# Autodesk Inventor assembly: робот - сборка фулл
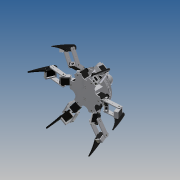
[picture p0: Inventor's stored thumbnail of the model, 180x180]
Saved by Autodesk Inventor 2020 (Build 240168000, 168)
## iProperties
Created: 2019-09-07
Part Number: робот - сборка фулл
Material: Типовые
Document SubType Name: Assembly
Designer: Iliga
Author: Iliga
## Documents named in this file (28)
- F:\GrabCAD\Robot\робот - сборка фулл.iam
- F:\GrabCAD\Robot\тело.ipt
- F:\GrabCAD\Robot\левая лапа - сборка.iam
- F:\GrabCAD\Robot\крепление2.ipt
- F:\GrabCAD\Robot\крепление-стенки.ipt
- F:\GrabCAD\Robot\полочка.ipt
- F:\GrabCAD\Robot\1.ipt
- F:\GrabCAD\Robot\Camera OV7670.iam
- F:\GrabCAD\Robot\28BYJ-48 – 5V Stepper Motor.ipt
- F:\GrabCAD\Robot\Крепление_двигатель малый.ipt
- F:\GrabCAD\Robot\Крепление_база.ipt
- F:\GrabCAD\Robot\Деталь1.ipt
- F:\GrabCAD\Robot\EN ISO 7045 - M4 x 8 - 4.8 - H(1).ipt
- F:\GrabCAD\Robot\EN ISO 7045 - M2 x 6 - 4.8 - H(1).ipt
- F:\GrabCAD\Robot\EN ISO 7045 - M1,6 x 4 - 4.8 - H(1).ipt
- F:\GrabCAD\Robot\EN ISO 7045 - M6 x 8 - 4.8 - H(1).ipt
- F:\GrabCAD\Robot\MP1584 Regulador.ipt
- F:\GrabCAD\Robot\Крепление Меги.ipt
- F:\GrabCAD\Robot\arduinoMegaDetailed.ipt
- F:\GrabCAD\Robot\Крепление батареек.ipt
- F:\GrabCAD\Robot\AAA_SIZE_BATTERY_CELL.ipt
- F:\GrabCAD\Robot\Bluetooth adapter крышка.ipt
- F:\GrabCAD\Robot\DC-DC корпус.ipt
- F:\GrabCAD\Robot\Bluetooth adapter корпус.ipt
- F:\GrabCAD\Robot\HM10.iam
- F:\GrabCAD\Robot\EN ISO 7045 - M3 x 6 - 4.8 - H(1).ipt
- F:\GrabCAD\Robot\ULN2003.ipt
- F:\GrabCAD\Robot\крепление_драйвера.ipt
## Components (135 placed, 25 different names)
1. лапа:1 [sub-assembly] — Совмещение:92, Совмещение:97, Совмещение:173, Совмещение:179
2. лапа:2 [sub-assembly] — Совмещение:89, Совмещение:91, Совмещение:175
3. лапа:3 [sub-assembly] — Совмещение:90, Совмещение:96
4. лапа:4 [sub-assembly] — Совмещение:159, Совмещение:160, Совмещение:178
5. лапа:5 [sub-assembly] — Совмещение:161, Совмещение:163
6. лапа:6 [sub-assembly] — Совмещение:162, Совмещение:164, Совмещение:176
7. крепление-стенки:1 — Совмещение:86, Совмещение:87, Совмещение:88, Совмещение:126, Совмещение:127, Совмещение:128
8. крепление2:1 — Совмещение:86, Совмещение:87, Совмещение:88, Совмещение:89, Совмещение:90, Совмещение:91, Совмещение:92, Совмещение:96, Совмещение:97, Совмещение:166, Совмещение:167, Совмещение:168, Совмещение:169, Совмещение:170, Совмещение:171, Совмещение:172, Допуск симметричности:1
9. тело основа:1 — Совмещение:49, Заподлицо:1, Касательность:1, Совмещение:118, Совмещение:132, Совмещение:184, Совмещение:185, Совмещение:186, Совмещение:187
10. тело основа:2 — Совмещение:49, Заподлицо:1, Касательность:1, Совмещение:120, Совмещение:121, Совмещение:122, Совмещение:123
11. тело основа:3 — Совмещение:120, Совмещение:121, Совмещение:122, Заподлицо:2, Совмещение:126, Совмещение:127, Совмещение:128, Совмещение:159, Совмещение:160, Совмещение:161, Совмещение:162, Совмещение:163, Совмещение:164, Допуск симметричности:1, Совмещение:173, Совмещение:175, Совмещение:176, Совмещение:178, Совмещение:179, Совмещение:180, Совмещение:181, Совмещение:182, Совмещение:183
12. полочка:1 — Совмещение:118, Совмещение:123, Заподлицо:2, Заподлицо:4, Совмещение:136, Совмещение:137, Совмещение:138, Совмещение:140, Совмещение:141, Совмещение:142, Совмещение:143, Совмещение:144, Совмещение:149, Совмещение:150, Совмещение:151, Совмещение:152, Совмещение:225, Совмещение:238, Совмещение:309, Совмещение:373, Совмещение:378, Совмещение:379, Совмещение:392, Совмещение:397, Совмещение:398, Совмещение:399, Совмещение:400, Совмещение:401, Совмещение:402, Совмещение:403, Совмещение:404, Совмещение:405, Совмещение:406, Совмещение:407, Совмещение:408, Совмещение:409, Совмещение:410, Совмещение:411, Совмещение:412, Совмещение:413, Совмещение:429, Совмещение:430, Совмещение:431, Совмещение:447, Совмещение:448, Совмещение:449, Совмещение:465, Совмещение:466, Совмещение:467
13. Camera OV7670:1 [sub-assembly] — Совмещение:156, Совмещение:165
14. 28BYJ-48 – 5V Stepper Motor:1 — Совмещение:131, Совмещение:132, Заподлицо:4, Совмещение:133, Совмещение:134, Совмещение:135, Совмещение:153, Совмещение:154, Совмещение:155
15. Крепление_двигатель малый:1 — Совмещение:133, Совмещение:134, Совмещение:135
16. Крепление:1 — Совмещение:137, Совмещение:141, Совмещение:142
17. Крепление:2 — Совмещение:136, Совмещение:138, Совмещение:140
18. Крепление:3 — Совмещение:144, Совмещение:151, Совмещение:152
19. Крепление:4 — Совмещение:143, Совмещение:149, Совмещение:150
20. Деталь1:1 — Совмещение:153, Совмещение:154, Совмещение:155, Совмещение:156, Совмещение:165
21. BS EN ISO 7045 H - метрическая M2 x 6 - 4.8 - H:9 — Заподлицо:8, Заподлицо:10
22. BS EN ISO 7045 H - метрическая M2 x 6 - 4.8 - H:10 — Заподлицо:8
23. BS EN ISO 7045 H - метрическая M2 x 6 - 4.8 - H:11 — Заподлицо:9, Заподлицо:10
24. BS EN ISO 7045 H - метрическая M2 x 6 - 4.8 - H:12 — Заподлицо:9
25. BS EN ISO 7045 H - метрическая M2 x 6 - 4.8 - H:13
26. BS EN ISO 7045 H - метрическая M2 x 6 - 4.8 - H:14
27. BS EN ISO 7045 H - метрическая M2 x 6 - 4.8 - H:15
28. BS EN ISO 7045 H - метрическая M2 x 6 - 4.8 - H:16
29. BS EN ISO 7045 H - метрическая M6 x 8 - 4.8 - H:1 — Совмещение:184, Совмещение:185
30. BS EN ISO 7045 H - метрическая M6 x 8 - 4.8 - H:2 — Совмещение:186, Совмещение:187
31. MP1584 Regulador:1 — Совмещение:208, Совмещение:209, Совмещение:210
32. Крепление Меги:1 — Совмещение:188, Совмещение:189, Совмещение:190, Совмещение:191, Совмещение:192, Совмещение:193
33. arduinoMegaDetailed:1 — Совмещение:188, Совмещение:189, Совмещение:190, Совмещение:239, Совмещение:240, Совмещение:241, Совмещение:242
34. Крепление батареек:1 — Совмещение:194, Совмещение:195, Совмещение:196, Совмещение:197, Совмещение:198, Совмещение:199, Совмещение:200, Совмещение:201
35. AAA_SIZE_BATTERY_CELL:1 — Совмещение:194, Заподлицо:15, Совмещение:198
36. AAA_SIZE_BATTERY_CELL:2 — Совмещение:195, Заподлицо:14, Заподлицо:15
37. AAA_SIZE_BATTERY_CELL:3 — Совмещение:196, Заподлицо:13, Заподлицо:14
38. AAA_SIZE_BATTERY_CELL:4 — Совмещение:197, Заподлицо:13
39. DC-DC крышка:1 — Совмещение:211, Совмещение:212, Заподлицо:16
40. DC-DC корпус:1 — Совмещение:208, Совмещение:209, Совмещение:210, Совмещение:211, Совмещение:212, Заподлицо:16, Совмещение:213, Совмещение:214, Совмещение:215, Совмещение:216, Совмещение:217, Совмещение:218, Совмещение:219, Совмещение:220, Совмещение:221, Совмещение:222, Совмещение:223, Совмещение:224
41. Крепление:13 — Совмещение:213, Совмещение:214, Совмещение:215, Совмещение:225
42. Крепление:14 — Совмещение:216, Совмещение:217, Совмещение:218
43. Крепление:15 — Совмещение:219, Совмещение:220, Совмещение:221, Совмещение:407, Совмещение:408
44. Крепление:16 — Совмещение:222, Совмещение:223, Совмещение:224
45. DC-DC корпус:2 — Совмещение:228, Совмещение:229, Совмещение:230, Заподлицо:17, Совмещение:231, Совмещение:232, Совмещение:233, Совмещение:234, Совмещение:235
46. DC-DC крышка:2 — Заподлицо:17, Совмещение:231, Совмещение:232
47. HM10:1 [sub-assembly] — Совмещение:228, Совмещение:229, Совмещение:230
48. BS EN ISO 7045 H - метрическая M3 x 6 - 4.8 - H:1 — Совмещение:241, Совмещение:242
49. BS EN ISO 7045 H - метрическая M3 x 6 - 4.8 - H:2 — Совмещение:239, Совмещение:240
50. ULN2003:1 — Совмещение:244, Совмещение:245, Совмещение:246
51. крепление_драйвера:1 — Совмещение:244, Совмещение:245, Совмещение:246, Совмещение:380, Совмещение:381, Совмещение:382, Совмещение:383, Совмещение:384, Совмещение:385, Совмещение:386, Совмещение:387, Совмещение:388, Совмещение:389, Совмещение:390, Совмещение:391
52. Крепление:21 — Совмещение:380, Совмещение:381, Совмещение:382
53. MP1584 Regulador:2
54. DC-DC корпус:3
55. Крепление:25
56. Крепление:26
57. Крепление:27 — Совмещение:309, Совмещение:409, Совмещение:410
58. Крепление:28
59. MP1584 Regulador:4
60. DC-DC корпус:5
61. Крепление:33
62. Крепление:34
63. Крепление:35 — Совмещение:411, Совмещение:412, Совмещение:413
64. Крепление:36
65. MP1584 Regulador:7
66. DC-DC корпус:8
67. Крепление:45
68. Крепление:46
69. Крепление:47 — Совмещение:405, Совмещение:406
70. Крепление:48 — Совмещение:373
71. Крепление:49 — Совмещение:383, Совмещение:384, Совмещение:385, Совмещение:392, Совмещение:400, Совмещение:401
72. Крепление:50 — Совмещение:386, Совмещение:387, Совмещение:388
73. Крепление:51 — Совмещение:389, Совмещение:390, Совмещение:391
74. MP1584 Regulador:8
75. DC-DC корпус:9
76. Крепление:52
77. Крепление:53
78. Крепление:54 — Совмещение:429, Совмещение:430, Совмещение:431
79. Крепление:55
80. MP1584 Regulador:9
81. DC-DC корпус:10
82. Крепление:56 — Совмещение:447
83. Крепление:57 — Совмещение:448, Совмещение:449
84. Крепление:58
85. Крепление:59
86. MP1584 Regulador:10
87. DC-DC корпус:11
88. Крепление:60
89. Крепление:61
90. Крепление:62 — Совмещение:465, Совмещение:466, Совмещение:467
91. Крепление:63
92. BS EN ISO 7045 H - метрическая M4 x 8 - 4.8 - H:1 — Совмещение:166, Совмещение:167
93. BS EN ISO 7045 H - метрическая M4 x 8 - 4.8 - H:2
94. BS EN ISO 7045 H - метрическая M4 x 8 - 4.8 - H:3
95. BS EN ISO 7045 H - метрическая M4 x 8 - 4.8 - H:4
96. BS EN ISO 7045 H - метрическая M4 x 8 - 4.8 - H:5
97. BS EN ISO 7045 H - метрическая M4 x 8 - 4.8 - H:6
98. BS EN ISO 7045 H - метрическая M2 x 6 - 4.8 - H:1 — Заподлицо:5, Заподлицо:6, Совмещение:171
99. BS EN ISO 7045 H - метрическая M2 x 6 - 4.8 - H:2 — Заподлицо:5, Совмещение:169, Совмещение:172
100. BS EN ISO 7045 H - метрическая M2 x 6 - 4.8 - H:4 — Заподлицо:6, Заподлицо:7, Совмещение:168
101. BS EN ISO 7045 H - метрическая M2 x 6 - 4.8 - H:3 — Заподлицо:7, Совмещение:170
102. BS EN ISO 7045 H - метрическая M2 x 6 - 4.8 - H:5
103. BS EN ISO 7045 H - метрическая M2 x 6 - 4.8 - H:6
104. BS EN ISO 7045 H - метрическая M2 x 6 - 4.8 - H:7
105. BS EN ISO 7045 H - метрическая M2 x 6 - 4.8 - H:8
106. BS EN ISO 7045 H - метрическая M1,6 x 4 - 4.8 - H:1 — Заподлицо:11, Совмещение:181
107. BS EN ISO 7045 H - метрическая M1,6 x 4 - 4.8 - H:3 — Заподлицо:11, Заподлицо:12, Совмещение:180
108. BS EN ISO 7045 H - метрическая M1,6 x 4 - 4.8 - H:2 — Заподлицо:12, Совмещение:182, Совмещение:183
109. BS EN ISO 7045 H - метрическая M1,6 x 4 - 4.8 - H:4
110. BS EN ISO 7045 H - метрическая M1,6 x 4 - 4.8 - H:5
111. BS EN ISO 7045 H - метрическая M1,6 x 4 - 4.8 - H:6
112. BS EN ISO 7045 H - метрическая M1,6 x 4 - 4.8 - H:7
113. BS EN ISO 7045 H - метрическая M1,6 x 4 - 4.8 - H:8
114. BS EN ISO 7045 H - метрическая M1,6 x 4 - 4.8 - H:9
115. BS EN ISO 7045 H - метрическая M1,6 x 4 - 4.8 - H:10
116. BS EN ISO 7045 H - метрическая M1,6 x 4 - 4.8 - H:11
117. BS EN ISO 7045 H - метрическая M1,6 x 4 - 4.8 - H:12
118. BS EN ISO 7045 H - метрическая M1,6 x 4 - 4.8 - H:13
119. BS EN ISO 7045 H - метрическая M1,6 x 4 - 4.8 - H:14
120. BS EN ISO 7045 H - метрическая M1,6 x 4 - 4.8 - H:15
121. BS EN ISO 7045 H - метрическая M1,6 x 4 - 4.8 - H:16
122. BS EN ISO 7045 H - метрическая M1,6 x 4 - 4.8 - H:17
123. BS EN ISO 7045 H - метрическая M1,6 x 4 - 4.8 - H:18
124. Крепление:5 — Совмещение:191, Совмещение:192, Совмещение:193, Совмещение:397, Совмещение:398, Совмещение:399
125. Крепление:6
126. Крепление:7
127. Крепление:8
128. Крепление:9 — Совмещение:199, Совмещение:200, Совмещение:201, Совмещение:402, Совмещение:403, Совмещение:404
129. Крепление:10
130. Крепление:11
131. Крепление:12
132. Крепление:17 — Совмещение:233, Совмещение:234, Совмещение:235, Совмещение:238, Совмещение:378, Совмещение:379
133. Крепление:18
134. Крепление:19
135. Крепление:20
## Component patterns: (6 elements, first: BS EN ISO 7045 H - метрическая M4 x 8 - 4.8 - H:1), (2 elements, first: BS EN ISO 7045 H - метрическая M2 x 6 - 4.8 - H:1 + BS EN ISO 7045 H - метрическая M2 x 6 - 4.8 - H:2 + BS EN ISO 7045 H - метрическая M2 x 6 - 4.8 - H:4 + BS EN ISO 7045 H - метрическая M2 x 6 - 4.8 - H:3), (6 elements, first: BS EN ISO 7045 H - метрическая M1,6 x 4 - 4.8 - H:1 + BS EN ISO 7045 H - метрическая M1,6 x 4 - 4.8 - H:3 + BS EN ISO 7045 H - метрическая M1,6 x 4 - 4.8 - H:2), (4 elements, first: Крепление:5), (4 elements, first: Крепление:9), (4 elements, first: Крепление:17)
## Relationships (265: Mate 247, Flush 16, Tangent 1, Symmetry 1)
- Совмещение:49 [Mate]: тело основа:1 ↔ тело основа:2
- Заподлицо:1 [Flush]: тело основа:1 ↔ тело основа:2
- Совмещение:86 [Mate]: крепление-стенки:1 ↔ крепление2:1
- Совмещение:87 [Mate]: крепление-стенки:1 ↔ крепление2:1
- Совмещение:88 [Mate]: крепление-стенки:1 ↔ крепление2:1
- Совмещение:89 [Mate]: лапа:2 ↔ крепление2:1
- Совмещение:90 [Mate]: лапа:3 ↔ крепление2:1
- Совмещение:91 [Mate]: лапа:2 ↔ крепление2:1
- Совмещение:92 [Mate]: лапа:1 ↔ крепление2:1
- Совмещение:96 [Mate]: лапа:3 ↔ крепление2:1
- Совмещение:97 [Mate]: лапа:1 ↔ крепление2:1
- Касательность:1 [Tangent]: тело основа:1 ↔ тело основа:2
- Совмещение:118 [Mate]: тело основа:1 ↔ полочка:1
- Совмещение:120 [Mate]: тело основа:2 ↔ тело основа:3
- Совмещение:121 [Mate]: тело основа:2 ↔ тело основа:3
- Совмещение:122 [Mate]: тело основа:2 ↔ тело основа:3
- Совмещение:123 [Mate]: тело основа:2 ↔ полочка:1
- Заподлицо:2 [Flush]: тело основа:3 ↔ полочка:1
- Совмещение:126 [Mate]: крепление-стенки:1 ↔ тело основа:3
- Совмещение:127 [Mate]: крепление-стенки:1 ↔ тело основа:3
- Совмещение:128 [Mate]: крепление-стенки:1 ↔ тело основа:3
- Совмещение:131 [Mate]: 28BYJ-48 – 5V Stepper Motor:1
- Совмещение:132 [Mate]: тело основа:1 ↔ 28BYJ-48 – 5V Stepper Motor:1
- Заподлицо:4 [Flush]: полочка:1 ↔ 28BYJ-48 – 5V Stepper Motor:1
- Совмещение:133 [Mate]: 28BYJ-48 – 5V Stepper Motor:1 ↔ Крепление_двигатель малый:1
- Совмещение:134 [Mate]: 28BYJ-48 – 5V Stepper Motor:1 ↔ Крепление_двигатель малый:1
- Совмещение:135 [Mate]: 28BYJ-48 – 5V Stepper Motor:1 ↔ Крепление_двигатель малый:1
- Совмещение:136 [Mate]: полочка:1 ↔ Крепление:2
- Совмещение:137 [Mate]: полочка:1 ↔ Крепление:1
- Совмещение:138 [Mate]: полочка:1 ↔ Крепление:2
- Совмещение:140 [Mate]: полочка:1 ↔ Крепление:2
- Совмещение:141 [Mate]: полочка:1 ↔ Крепление:1
- Совмещение:142 [Mate]: полочка:1 ↔ Крепление:1
- Совмещение:143 [Mate]: полочка:1 ↔ Крепление:4
- Совмещение:144 [Mate]: полочка:1 ↔ Крепление:3
- Совмещение:149 [Mate]: полочка:1 ↔ Крепление:4
- Совмещение:150 [Mate]: полочка:1 ↔ Крепление:4
- Совмещение:151 [Mate]: полочка:1 ↔ Крепление:3
- Совмещение:152 [Mate]: полочка:1 ↔ Крепление:3
- Совмещение:153 [Mate]: 28BYJ-48 – 5V Stepper Motor:1 ↔ Деталь1:1
- Совмещение:154 [Mate] (0.1 mm): 28BYJ-48 – 5V Stepper Motor:1 ↔ Деталь1:1
- Совмещение:155 [Mate]: 28BYJ-48 – 5V Stepper Motor:1 ↔ Деталь1:1
- Совмещение:156 [Mate]: Camera OV7670:1 ↔ Деталь1:1
- Совмещение:159 [Mate]: лапа:4 ↔ тело основа:3
- Совмещение:160 [Mate]: лапа:4 ↔ тело основа:3
- Совмещение:161 [Mate]: лапа:5 ↔ тело основа:3
- Совмещение:162 [Mate]: лапа:6 ↔ тело основа:3
- Совмещение:163 [Mate]: лапа:5 ↔ тело основа:3
- Совмещение:164 [Mate]: лапа:6 ↔ тело основа:3
- Совмещение:165 [Mate]: Camera OV7670:1 ↔ Деталь1:1
- Совмещение:166 [Mate]: крепление2:1 ↔ BS EN ISO 7045 H - метрическая M4 x 8 - 4.8 - H:1
- Совмещение:167 [Mate]: крепление2:1 ↔ BS EN ISO 7045 H - метрическая M4 x 8 - 4.8 - H:1
- Заподлицо:5 [Flush]: BS EN ISO 7045 H - метрическая M2 x 6 - 4.8 - H:1 ↔ BS EN ISO 7045 H - метрическая M2 x 6 - 4.8 - H:2
- Заподлицо:6 [Flush]: BS EN ISO 7045 H - метрическая M2 x 6 - 4.8 - H:1 ↔ BS EN ISO 7045 H - метрическая M2 x 6 - 4.8 - H:4
- Заподлицо:7 [Flush]: BS EN ISO 7045 H - метрическая M2 x 6 - 4.8 - H:4 ↔ BS EN ISO 7045 H - метрическая M2 x 6 - 4.8 - H:3
- Совмещение:168 [Mate]: крепление2:1 ↔ BS EN ISO 7045 H - метрическая M2 x 6 - 4.8 - H:4
- Совмещение:169 [Mate]: крепление2:1 ↔ BS EN ISO 7045 H - метрическая M2 x 6 - 4.8 - H:2
- Совмещение:170 [Mate]: крепление2:1 ↔ BS EN ISO 7045 H - метрическая M2 x 6 - 4.8 - H:3
- Совмещение:171 [Mate]: крепление2:1 ↔ BS EN ISO 7045 H - метрическая M2 x 6 - 4.8 - H:1
- Совмещение:172 [Mate]: крепление2:1 ↔ BS EN ISO 7045 H - метрическая M2 x 6 - 4.8 - H:2
- Допуск симметричности:1 [Symmetry]: крепление2:1 ↔ тело основа:3
- Заподлицо:8 [Flush]: BS EN ISO 7045 H - метрическая M2 x 6 - 4.8 - H:9 ↔ BS EN ISO 7045 H - метрическая M2 x 6 - 4.8 - H:10
- Заподлицо:9 [Flush]: BS EN ISO 7045 H - метрическая M2 x 6 - 4.8 - H:11 ↔ BS EN ISO 7045 H - метрическая M2 x 6 - 4.8 - H:12
- Заподлицо:10 [Flush]: BS EN ISO 7045 H - метрическая M2 x 6 - 4.8 - H:9 ↔ BS EN ISO 7045 H - метрическая M2 x 6 - 4.8 - H:11
- Совмещение:173 [Mate]: лапа:1 ↔ тело основа:3
- Совмещение:175 [Mate]: лапа:2 ↔ тело основа:3
- Совмещение:176 [Mate]: лапа:6 ↔ тело основа:3
- Совмещение:178 [Mate]: лапа:4 ↔ тело основа:3
- Совмещение:179 [Mate]: лапа:1 ↔ тело основа:3
- Заподлицо:11 [Flush]: BS EN ISO 7045 H - метрическая M1,6 x 4 - 4.8 - H:1 ↔ BS EN ISO 7045 H - метрическая M1,6 x 4 - 4.8 - H:3
- Заподлицо:12 [Flush]: BS EN ISO 7045 H - метрическая M1,6 x 4 - 4.8 - H:3 ↔ BS EN ISO 7045 H - метрическая M1,6 x 4 - 4.8 - H:2
- Совмещение:180 [Mate]: тело основа:3 ↔ BS EN ISO 7045 H - метрическая M1,6 x 4 - 4.8 - H:3
- Совмещение:181 [Mate]: тело основа:3 ↔ BS EN ISO 7045 H - метрическая M1,6 x 4 - 4.8 - H:1
- Совмещение:182 [Mate]: тело основа:3 ↔ BS EN ISO 7045 H - метрическая M1,6 x 4 - 4.8 - H:2
- Совмещение:183 [Mate]: тело основа:3 ↔ BS EN ISO 7045 H - метрическая M1,6 x 4 - 4.8 - H:2
- Совмещение:184 [Mate]: тело основа:1 ↔ BS EN ISO 7045 H - метрическая M6 x 8 - 4.8 - H:1
- Совмещение:185 [Mate]: тело основа:1 ↔ BS EN ISO 7045 H - метрическая M6 x 8 - 4.8 - H:1
- Совмещение:186 [Mate]: тело основа:1 ↔ BS EN ISO 7045 H - метрическая M6 x 8 - 4.8 - H:2
- Совмещение:187 [Mate]: тело основа:1 ↔ BS EN ISO 7045 H - метрическая M6 x 8 - 4.8 - H:2
- Совмещение:188 [Mate]: Крепление Меги:1 ↔ arduinoMegaDetailed:1
- Совмещение:189 [Mate]: Крепление Меги:1 ↔ arduinoMegaDetailed:1
- Совмещение:190 [Mate]: Крепление Меги:1 ↔ arduinoMegaDetailed:1
- Совмещение:191 [Mate]: Крепление Меги:1 ↔ Крепление:5
- Совмещение:192 [Mate]: Крепление Меги:1 ↔ Крепление:5
- Совмещение:193 [Mate]: Крепление Меги:1 ↔ Крепление:5
- Совмещение:194 [Mate]: Крепление батареек:1 ↔ AAA_SIZE_BATTERY_CELL:1
- Совмещение:195 [Mate]: Крепление батареек:1 ↔ AAA_SIZE_BATTERY_CELL:2
- Совмещение:196 [Mate]: Крепление батареек:1 ↔ AAA_SIZE_BATTERY_CELL:3
- Совмещение:197 [Mate]: Крепление батареек:1 ↔ AAA_SIZE_BATTERY_CELL:4
- Заподлицо:13 [Flush]: AAA_SIZE_BATTERY_CELL:3 ↔ AAA_SIZE_BATTERY_CELL:4
- Заподлицо:14 [Flush]: AAA_SIZE_BATTERY_CELL:2 ↔ AAA_SIZE_BATTERY_CELL:3
- Заподлицо:15 [Flush]: AAA_SIZE_BATTERY_CELL:1 ↔ AAA_SIZE_BATTERY_CELL:2
- Совмещение:198 [Mate]: Крепление батареек:1 ↔ AAA_SIZE_BATTERY_CELL:1
- Совмещение:199 [Mate]: Крепление батареек:1 ↔ Крепление:9
- Совмещение:200 [Mate]: Крепление батареек:1 ↔ Крепление:9
- Совмещение:201 [Mate]: Крепление батареек:1 ↔ Крепление:9
- Совмещение:208 [Mate]: MP1584 Regulador:1 ↔ DC-DC корпус:1
- Совмещение:209 [Mate]: MP1584 Regulador:1 ↔ DC-DC корпус:1
- Совмещение:210 [Mate]: MP1584 Regulador:1 ↔ DC-DC корпус:1
- Совмещение:211 [Mate]: DC-DC крышка:1 ↔ DC-DC корпус:1
- Совмещение:212 [Mate]: DC-DC крышка:1 ↔ DC-DC корпус:1
- Заподлицо:16 [Flush]: DC-DC крышка:1 ↔ DC-DC корпус:1
- Совмещение:213 [Mate]: DC-DC корпус:1 ↔ Крепление:13
- Совмещение:214 [Mate]: DC-DC корпус:1 ↔ Крепление:13
- Совмещение:215 [Mate]: DC-DC корпус:1 ↔ Крепление:13
- Совмещение:216 [Mate]: DC-DC корпус:1 ↔ Крепление:14
- Совмещение:217 [Mate]: DC-DC корпус:1 ↔ Крепление:14
- Совмещение:218 [Mate]: DC-DC корпус:1 ↔ Крепление:14
- Совмещение:219 [Mate]: DC-DC корпус:1 ↔ Крепление:15
- Совмещение:220 [Mate]: DC-DC корпус:1 ↔ Крепление:15
- Совмещение:221 [Mate]: DC-DC корпус:1 ↔ Крепление:15
- Совмещение:222 [Mate]: DC-DC корпус:1 ↔ Крепление:16
- Совмещение:223 [Mate]: DC-DC корпус:1 ↔ Крепление:16
- Совмещение:224 [Mate]: DC-DC корпус:1 ↔ Крепление:16
- Совмещение:225 [Mate]: полочка:1 ↔ Крепление:13
- Совмещение:228 [Mate]: DC-DC корпус:2 ↔ HM10:1
- Совмещение:229 [Mate]: DC-DC корпус:2 ↔ HM10:1
- Совмещение:230 [Mate]: DC-DC корпус:2 ↔ HM10:1
- Заподлицо:17 [Flush]: DC-DC корпус:2 ↔ DC-DC крышка:2
- Совмещение:231 [Mate]: DC-DC корпус:2 ↔ DC-DC крышка:2
- Совмещение:232 [Mate]: DC-DC корпус:2 ↔ DC-DC крышка:2
- Совмещение:233 [Mate]: DC-DC корпус:2 ↔ Крепление:17
- Совмещение:234 [Mate]: DC-DC корпус:2 ↔ Крепление:17
- Совмещение:235 [Mate]: DC-DC корпус:2 ↔ Крепление:17
- Совмещение:238 [Mate]: полочка:1 ↔ Крепление:17
- Совмещение:239 [Mate]: arduinoMegaDetailed:1 ↔ BS EN ISO 7045 H - метрическая M3 x 6 - 4.8 - H:2
- Совмещение:240 [Mate]: arduinoMegaDetailed:1 ↔ BS EN ISO 7045 H - метрическая M3 x 6 - 4.8 - H:2
- Совмещение:241 [Mate]: arduinoMegaDetailed:1 ↔ BS EN ISO 7045 H - метрическая M3 x 6 - 4.8 - H:1
- Совмещение:242 [Mate]: arduinoMegaDetailed:1 ↔ BS EN ISO 7045 H - метрическая M3 x 6 - 4.8 - H:1
- Совмещение:244 [Mate]: ULN2003:1 ↔ крепление_драйвера:1
- Совмещение:245 [Mate]: ULN2003:1 ↔ крепление_драйвера:1
- Совмещение:246 [Mate]: ULN2003:1 ↔ крепление_драйвера:1
- [Mate]: MP1584 Regulador:2 ↔ DC-DC корпус:3
- [Mate]: MP1584 Regulador:2 ↔ DC-DC корпус:3
- [Mate]: MP1584 Regulador:2 ↔ DC-DC корпус:3
- [Mate]: DC-DC корпус:3 ↔ Крепление:25
- [Mate]: DC-DC корпус:3 ↔ Крепление:25
- [Mate]: DC-DC корпус:3 ↔ Крепление:25
- [Mate]: DC-DC корпус:3 ↔ Крепление:26
- [Mate]: DC-DC корпус:3 ↔ Крепление:26
- [Mate]: DC-DC корпус:3 ↔ Крепление:26
- [Mate]: DC-DC корпус:3 ↔ Крепление:27
- [Mate]: DC-DC корпус:3 ↔ Крепление:27
- [Mate]: DC-DC корпус:3 ↔ Крепление:27
- [Mate]: DC-DC корпус:3 ↔ Крепление:28
- [Mate]: DC-DC корпус:3 ↔ Крепление:28
- [Mate]: DC-DC корпус:3 ↔ Крепление:28
- [Mate]: MP1584 Regulador:4 ↔ DC-DC корпус:5
- [Mate]: MP1584 Regulador:4 ↔ DC-DC корпус:5
- [Mate]: MP1584 Regulador:4 ↔ DC-DC корпус:5
- [Mate]: DC-DC корпус:5 ↔ Крепление:33
- [Mate]: DC-DC корпус:5 ↔ Крепление:33
- [Mate]: DC-DC корпус:5 ↔ Крепление:33
- [Mate]: DC-DC корпус:5 ↔ Крепление:34
- [Mate]: DC-DC корпус:5 ↔ Крепление:34
- [Mate]: DC-DC корпус:5 ↔ Крепление:34
- [Mate]: DC-DC корпус:5 ↔ Крепление:35
- [Mate]: DC-DC корпус:5 ↔ Крепление:35
- [Mate]: DC-DC корпус:5 ↔ Крепление:35
- [Mate]: DC-DC корпус:5 ↔ Крепление:36
- [Mate]: DC-DC корпус:5 ↔ Крепление:36
- [Mate]: DC-DC корпус:5 ↔ Крепление:36
- Совмещение:309 [Mate]: полочка:1 ↔ Крепление:27
- [Mate]: MP1584 Regulador:7 ↔ DC-DC корпус:8
- [Mate]: MP1584 Regulador:7 ↔ DC-DC корпус:8
- [Mate]: MP1584 Regulador:7 ↔ DC-DC корпус:8
- [Mate]: DC-DC корпус:8 ↔ Крепление:45
- [Mate]: DC-DC корпус:8 ↔ Крепление:45
- [Mate]: DC-DC корпус:8 ↔ Крепление:45
- [Mate]: DC-DC корпус:8 ↔ Крепление:46
- [Mate]: DC-DC корпус:8 ↔ Крепление:46
- [Mate]: DC-DC корпус:8 ↔ Крепление:46
- [Mate]: DC-DC корпус:8 ↔ Крепление:47
- [Mate]: DC-DC корпус:8 ↔ Крепление:47
- [Mate]: DC-DC корпус:8 ↔ Крепление:47
- [Mate]: DC-DC корпус:8 ↔ Крепление:48
- [Mate]: DC-DC корпус:8 ↔ Крепление:48
- [Mate]: DC-DC корпус:8 ↔ Крепление:48
- Совмещение:373 [Mate]: полочка:1 ↔ Крепление:48
- Совмещение:378 [Mate]: полочка:1 ↔ Крепление:17
- Совмещение:379 [Mate]: полочка:1 ↔ Крепление:17
- Совмещение:380 [Mate]: крепление_драйвера:1 ↔ Крепление:21
- Совмещение:381 [Mate]: крепление_драйвера:1 ↔ Крепление:21
- Совмещение:382 [Mate]: крепление_драйвера:1 ↔ Крепление:21
- Совмещение:383 [Mate]: крепление_драйвера:1 ↔ Крепление:49
- Совмещение:384 [Mate]: крепление_драйвера:1 ↔ Крепление:49
- Совмещение:385 [Mate]: крепление_драйвера:1 ↔ Крепление:49
- Совмещение:386 [Mate]: крепление_драйвера:1 ↔ Крепление:50
- Совмещение:387 [Mate]: крепление_драйвера:1 ↔ Крепление:50
- Совмещение:388 [Mate]: крепление_драйвера:1 ↔ Крепление:50
- Совмещение:389 [Mate]: крепление_драйвера:1 ↔ Крепление:51
- Совмещение:390 [Mate]: крепление_драйвера:1 ↔ Крепление:51
- Совмещение:391 [Mate]: крепление_драйвера:1 ↔ Крепление:51
- Совмещение:392 [Mate]: полочка:1 ↔ Крепление:49
- Совмещение:397 [Mate]: полочка:1 ↔ Крепление:5
- Совмещение:398 [Mate]: полочка:1 ↔ Крепление:5
- Совмещение:399 [Mate]: полочка:1 ↔ Крепление:5
- Совмещение:400 [Mate]: полочка:1 ↔ Крепление:49
- Совмещение:401 [Mate]: полочка:1 ↔ Крепление:49
- Совмещение:402 [Mate]: полочка:1 ↔ Крепление:9
- Совмещение:403 [Mate]: полочка:1 ↔ Крепление:9
- Совмещение:404 [Mate]: полочка:1 ↔ Крепление:9
- Совмещение:405 [Mate]: полочка:1 ↔ Крепление:47
- Совмещение:406 [Mate]: полочка:1 ↔ Крепление:47
- Совмещение:407 [Mate]: полочка:1 ↔ Крепление:15
- Совмещение:408 [Mate]: полочка:1 ↔ Крепление:15
- Совмещение:409 [Mate]: полочка:1 ↔ Крепление:27
- Совмещение:410 [Mate]: полочка:1 ↔ Крепление:27
- Совмещение:411 [Mate]: полочка:1 ↔ Крепление:35
- Совмещение:412 [Mate]: полочка:1 ↔ Крепление:35
- Совмещение:413 [Mate]: полочка:1 ↔ Крепление:35
- [Mate]: MP1584 Regulador:8 ↔ DC-DC корпус:9
- [Mate]: MP1584 Regulador:8 ↔ DC-DC корпус:9
- [Mate]: MP1584 Regulador:8 ↔ DC-DC корпус:9
- [Mate]: DC-DC корпус:9 ↔ Крепление:52
- [Mate]: DC-DC корпус:9 ↔ Крепление:52
- [Mate]: DC-DC корпус:9 ↔ Крепление:52
- [Mate]: DC-DC корпус:9 ↔ Крепление:53
- [Mate]: DC-DC корпус:9 ↔ Крепление:53
- [Mate]: DC-DC корпус:9 ↔ Крепление:53
- [Mate]: DC-DC корпус:9 ↔ Крепление:54
- [Mate]: DC-DC корпус:9 ↔ Крепление:54
- [Mate]: DC-DC корпус:9 ↔ Крепление:54
- [Mate]: DC-DC корпус:9 ↔ Крепление:55
- [Mate]: DC-DC корпус:9 ↔ Крепление:55
- [Mate]: DC-DC корпус:9 ↔ Крепление:55
- Совмещение:429 [Mate]: полочка:1 ↔ Крепление:54
- Совмещение:430 [Mate]: полочка:1 ↔ Крепление:54
- Совмещение:431 [Mate]: полочка:1 ↔ Крепление:54
- [Mate]: MP1584 Regulador:9 ↔ DC-DC корпус:10
- [Mate]: MP1584 Regulador:9 ↔ DC-DC корпус:10
- [Mate]: MP1584 Regulador:9 ↔ DC-DC корпус:10
- [Mate]: DC-DC корпус:10 ↔ Крепление:56
- [Mate]: DC-DC корпус:10 ↔ Крепление:56
- [Mate]: DC-DC корпус:10 ↔ Крепление:56
- [Mate]: DC-DC корпус:10 ↔ Крепление:57
- [Mate]: DC-DC корпус:10 ↔ Крепление:57
- [Mate]: DC-DC корпус:10 ↔ Крепление:57
- [Mate]: DC-DC корпус:10 ↔ Крепление:58
- [Mate]: DC-DC корпус:10 ↔ Крепление:58
- [Mate]: DC-DC корпус:10 ↔ Крепление:58
- [Mate]: DC-DC корпус:10 ↔ Крепление:59
- [Mate]: DC-DC корпус:10 ↔ Крепление:59
- [Mate]: DC-DC корпус:10 ↔ Крепление:59
- Совмещение:447 [Mate]: полочка:1 ↔ Крепление:56
- Совмещение:448 [Mate]: полочка:1 ↔ Крепление:57
- Совмещение:449 [Mate]: полочка:1 ↔ Крепление:57
- [Mate]: MP1584 Regulador:10 ↔ DC-DC корпус:11
- [Mate]: MP1584 Regulador:10 ↔ DC-DC корпус:11
- [Mate]: MP1584 Regulador:10 ↔ DC-DC корпус:11
- [Mate]: DC-DC корпус:11 ↔ Крепление:60
- [Mate]: DC-DC корпус:11 ↔ Крепление:60
- [Mate]: DC-DC корпус:11 ↔ Крепление:60
- [Mate]: DC-DC корпус:11 ↔ Крепление:61
- [Mate]: DC-DC корпус:11 ↔ Крепление:61
- [Mate]: DC-DC корпус:11 ↔ Крепление:61
- [Mate]: DC-DC корпус:11 ↔ Крепление:62
- [Mate]: DC-DC корпус:11 ↔ Крепление:62
- [Mate]: DC-DC корпус:11 ↔ Крепление:62
- [Mate]: DC-DC корпус:11 ↔ Крепление:63
- [Mate]: DC-DC корпус:11 ↔ Крепление:63
- [Mate]: DC-DC корпус:11 ↔ Крепление:63
- Совмещение:465 [Mate]: полочка:1 ↔ Крепление:62
- Совмещение:466 [Mate]: полочка:1 ↔ Крепление:62
- Совмещение:467 [Mate]: полочка:1 ↔ Крепление:62
## Named parameters: d357_d308 = 0 mm, d358_d309 = 0 mm, d359_d310 = 0 mm, d360_d311 = 0 mm, d361_d312 = 0 mm, d362_d313 = 0 mm, d363_d314 = 0 mm, d364_d315 = 0 mm, d365_d316 = 0 mm, d366_d317 = 0 mm, d367_d300 = 0 mm, d368_d301 = 0 mm, d369_d302 = 0 mm, d370_d306 = 0 mm, d371_d307 = 0 mm, d387_d308 = 0 mm, d388_d309 = 0 mm, d389_d310 = 0 mm, d390_d311 = 0 mm, d391_d312 = 0 mm, d392_d313 = 0 mm, d393_d314 = 0 mm, d394_d315 = 0 mm, d395_d316 = 0 mm, d396_d317 = 0 mm, d397_d300 = 0 mm, d398_d301 = 0 mm, d399_d302 = 0 mm, d400_d306 = 0 mm, d401_d307 = 0 mm, d462_d372_d308 = 0 mm, d463_d373_d309 = 0 mm, d464_d374_d310 = 0 mm, d465_d375_d311 = 0 mm, d466_d376_d312 = 0 mm, d467_d377_d313 = 0 mm, d468_d378_d314 = 0 mm, d469_d379_d315 = 0 mm, d470_d380_d316 = 0 mm, d471_d381_d317 = 0 mm, d472_d382_d300 = 0 mm, d473_d383_d301 = 0 mm, d474_d384_d302 = 0 mm, d475_d385_d306 = 0 mm, d476_d386_d307 = 0 mm, d528_d387_d308 = 0 mm, d529_d388_d309 = 0 mm, d530_d389_d310 = 0 mm, d531_d390_d311 = 0 mm, d532_d391_d312 = 0 mm, d533_d392_d313 = 0 mm, d534_d393_d314 = 0 mm, d535_d394_d315 = 0 mm, d536_d395_d316 = 0 mm, d537_d396_d317 = 0 mm, d538_d397_d300 = 0 mm, d539_d398_d301 = 0 mm, d540_d399_d302 = 0 mm, d541_d400_d306 = 0 mm, d542_d401_d307 = 0 mm, d546_d387_d308 = 0 mm, d547_d388_d309 = 0 mm, d548_d389_d310 = 0 mm, d549_d390_d311 = 0 mm, d550_d391_d312 = 0 mm, d551_d392_d313 = 0 mm, d552_d393_d314 = 0 mm, d553_d394_d315 = 0 mm, d554_d395_d316 = 0 mm, d555_d396_d317 = 0 mm, d556_d397_d300 = 0 mm, d557_d398_d301 = 0 mm, d558_d399_d302 = 0 mm, d559_d400_d306 = 0 mm, d560_d401_d307 = 0 mm, d564_d546_d387_d308 = 0 mm, d565_d547_d388_d309 = 0 mm, d566_d548_d389_d310 = 0 mm, d567_d549_d390_d311 = 0 mm, d568_d550_d391_d312 = 0 mm, d569_d551_d392_d313 = 0 mm, d570_d552_d393_d314 = 0 mm, d571_d553_d394_d315 = 0 mm, d572_d554_d395_d316 = 0 mm, d573_d555_d396_d317 = 0 mm, d574_d556_d397_d300 = 0 mm, d575_d557_d398_d301 = 0 mm, d576_d558_d399_d302 = 0 mm, d577_d559_d400_d306 = 0 mm, d578_d560_d401_d307 = 0 mm
